# Autodesk Inventor assembly: BG002_trajan20_21
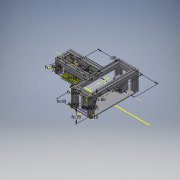
[picture p0: Inventor's stored thumbnail of the model, 180x180]
Saved by Autodesk Inventor 2022.2 (Build 262287000, 287)
## iProperties
Company: HTBLA Kaindorf
RuleStatus: InUse
Created: 2022-06-07
Part Number: BG002_trajan20_21
Project: Zeichenmaschine_v2
Material: Generisch
Description: eingebaute Motor
Document SubType Name: Assembly
Designer: trajan20
AfterDocNew0: iProperties-Editor_aufrufen
Author: jan
Keywords: 2021
## Documents named in this file (8)
- C:\Users\jan\Documents\DrawMachine\DrawMachineConstruction\Projekt\Zeichenmaschine_v2\BG002_trajan20_21_Zeichenmaschine_v2_eingebaute Motor.iam
- C:\Users\jan\Documents\DrawMachine\DrawMachineConstruction\Projekt\Zeichenmaschine_v2\BG001_trajan20_21_Zeichenmaschine_v2_Gerüst.iam
- C:\Users\jan\Documents\DrawMachine\DrawMachineConstruction\Projekt\Zeichenmaschine_v2\BT001_trajan20_21_Zeichenmaschine_v2_HauptPlatte.ipt
- C:\Users\jan\Documents\DrawMachine\DrawMachineConstruction\Projekt\Zeichenmaschine_v2\NEMA17_17HS19-2004S1_Stepperonline.ipt
- C:\Users\jan\Documents\DrawMachine\DrawMachineConstruction\Projekt\Zeichenmaschine_v2\BT002_trajan20_21_Zeichenmaschine_v2_GM_Platte.ipt
- C:\Users\jan\Documents\DrawMachine\DrawMachineConstruction\Projekt\Zeichenmaschine_v2\CUI_VGS-100B-12.ipt
- C:\Users\jan\Documents\DrawMachine\DrawMachineConstruction\Projekt\Zeichenmaschine_v2\BG005_trajan20_21_Zeichenmaschine_v2_winkel.iam
- C:\Users\jan\Documents\DrawMachine\DrawMachineConstruction\Projekt\Zeichenmaschine_v2\MISUMI_HBLBS5\AIS2022\HBLBS5.iam
## Components (8 placed, 7 different names)
1. BG001_trajan20_21_Zeichenmaschine_v2_Gerüst:1 [sub-assembly] — Fluchtend:1, Fluchtend:2, Passend:1, Fluchtend:3, Fluchtend:4, Passend:8, Passend:10, Fluchtend:6, Passend:12, Passend:13, Passend:14
2. BT001_trajan20_21_Zeichenmaschine_v2_HauptPlatte:1 — Fluchtend:1, Fluchtend:2, Passend:1, Passend:2, Passend:3, Passend:4, Passend:5, Passend:6, Passend:7, Passend:11
3. NEMA17_17HS19-2004S1_Stepperonline:1 — Passend:2, Passend:5, Passend:6
4. NEMA17_17HS19-2004S1_Stepperonline:2 — Passend:3, Passend:4, Passend:7
5. BT002_trajan20_21_Zeichenmaschine_v2_GM_Platte:1 — Fluchtend:3, Fluchtend:4, Passend:8
6. BG005_trajan20_21_Zeichenmaschine_v2_winkel:1 [sub-assembly] — Passend:10, Passend:11, Fluchtend:6
7. HBLBS5:1 [sub-assembly] — Passend:12, Passend:13
8. CUI_VGS-100B-12:1 — Passend:14
## Relationships (18: Mate 13, Flush 5)
- Fluchtend:1 [Flush]: BG001_trajan20_21_Zeichenmaschine_v2_Gerüst:1 ↔ BT001_trajan20_21_Zeichenmaschine_v2_HauptPlatte:1
- Fluchtend:2 [Flush]: BG001_trajan20_21_Zeichenmaschine_v2_Gerüst:1 ↔ BT001_trajan20_21_Zeichenmaschine_v2_HauptPlatte:1
- Passend:1 [Mate]: BG001_trajan20_21_Zeichenmaschine_v2_Gerüst:1 ↔ BT001_trajan20_21_Zeichenmaschine_v2_HauptPlatte:1
- Passend:2 [Mate]: BT001_trajan20_21_Zeichenmaschine_v2_HauptPlatte:1 ↔ NEMA17_17HS19-2004S1_Stepperonline:1
- Passend:3 [Mate]: BT001_trajan20_21_Zeichenmaschine_v2_HauptPlatte:1 ↔ NEMA17_17HS19-2004S1_Stepperonline:2
- Passend:4 [Mate]: BT001_trajan20_21_Zeichenmaschine_v2_HauptPlatte:1 ↔ NEMA17_17HS19-2004S1_Stepperonline:2
- Passend:5 [Mate]: BT001_trajan20_21_Zeichenmaschine_v2_HauptPlatte:1 ↔ NEMA17_17HS19-2004S1_Stepperonline:1
- Passend:6 [Mate]: BT001_trajan20_21_Zeichenmaschine_v2_HauptPlatte:1 ↔ NEMA17_17HS19-2004S1_Stepperonline:1
- Passend:7 [Mate]: BT001_trajan20_21_Zeichenmaschine_v2_HauptPlatte:1 ↔ NEMA17_17HS19-2004S1_Stepperonline:2
- Fluchtend:3 [Flush]: BG001_trajan20_21_Zeichenmaschine_v2_Gerüst:1 ↔ BT002_trajan20_21_Zeichenmaschine_v2_GM_Platte:1
- Fluchtend:4 [Flush]: BG001_trajan20_21_Zeichenmaschine_v2_Gerüst:1 ↔ BT002_trajan20_21_Zeichenmaschine_v2_GM_Platte:1
- Passend:8 [Mate]: BG001_trajan20_21_Zeichenmaschine_v2_Gerüst:1 ↔ BT002_trajan20_21_Zeichenmaschine_v2_GM_Platte:1
- Passend:10 [Mate]: BG001_trajan20_21_Zeichenmaschine_v2_Gerüst:1 ↔ BG005_trajan20_21_Zeichenmaschine_v2_winkel:1
- Passend:11 [Mate]: BT001_trajan20_21_Zeichenmaschine_v2_HauptPlatte:1 ↔ BG005_trajan20_21_Zeichenmaschine_v2_winkel:1
- Fluchtend:6 [Flush] (-5 mm): BG001_trajan20_21_Zeichenmaschine_v2_Gerüst:1 ↔ BG005_trajan20_21_Zeichenmaschine_v2_winkel:1
- Passend:12 [Mate]: BG001_trajan20_21_Zeichenmaschine_v2_Gerüst:1 ↔ HBLBS5:1
- Passend:13 [Mate] (-20 mm): BG001_trajan20_21_Zeichenmaschine_v2_Gerüst:1 ↔ HBLBS5:1
- Passend:14 [Mate]: BG001_trajan20_21_Zeichenmaschine_v2_Gerüst:1 ↔ CUI_VGS-100B-12:1
